# Autodesk Inventor assembly: coupler extention arm collector bottom
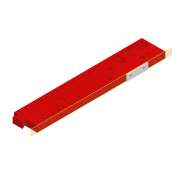
[picture p0: Inventor's stored thumbnail of the model, 180x180]
Saved by Autodesk Inventor 2020 (Build 240168000, 168)
## iProperties
Created: 2019-12-31
Part Number: coupler extention arm collector bottom
Document SubType Name: Assembly
Designer: ball
Author: ball
## Documents named in this file (4)
- C:\FTC\FTC8863CAD\2019 Robot\Delivery\extension arm\coupler extention arm collector bottom.iam
- C:\FTC\FTC8863CAD\2019 Robot\Collection\Collection rotation adapter.ipt
- C:\FTC\FTC8863CAD\2019 Robot\Delivery\extension arm\Coupler extension arm short edited holes for servo.ipt
- C:\FTC\FTC8863CAD\2019 Robot\Delivery\extension arm\standoff for gripper servo.ipt
## Components (3 placed, 3 different names)
1. Collection rotation adapter:1 — Mate:1, Mate:2, Mate:3
2. Coupler extension arm short edited holes for servo:1 — Mate:1, Mate:2, Mate:3, Flush:1, Flush:2
3. standoff for gripper servo:1 — Flush:1, Flush:2
## Relationships (5: Mate 3, Flush 2)
- Mate:1: Collection rotation adapter:1 ↔ Coupler extension arm short edited holes for servo:1
- Mate:2: Collection rotation adapter:1 ↔ Coupler extension arm short edited holes for servo:1
- Mate:3: Collection rotation adapter:1 ↔ Coupler extension arm short edited holes for servo:1
- Flush:1: Coupler extension arm short edited holes for servo:1 ↔ standoff for gripper servo:1
- Flush:2: Coupler extension arm short edited holes for servo:1 ↔ standoff for gripper servo:1
